# Autodesk Inventor assembly: Servo-Arm-52mm-Ball-Joint
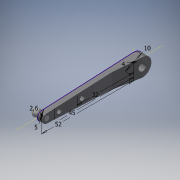
[picture p0: Inventor's stored thumbnail of the model, 180x180]
Saved by Autodesk Inventor 2018.2 (Build 222227000, 227)
## iProperties
Created: 2018-02-18
Part Number: Servo-Arm-52mm-Ball-Joint
Material: Generisch
Document SubType Name: Assembly
Designer: JochenAlt
Author: JochenAlt
## Documents named in this file (3)
- D:\Projects\Donna\CAD\Servo-Arm-52mm-Ball-Joint.iam
- D:\Projects\Donna\CAD\Ball-Joint-male.ipt
- D:\Projects\Donna\CAD\Servo-Arm-52mm.ipt
## Components (2 placed, 2 different names)
1. ball joint:1 — Passend:1, Passend:2
2. ServoArm:2 — Passend:1, Passend:2, Passend:3, Passend:4, Passend:5, Passend:6
## Relationships (6: Mate 6)
- Passend:1 [Mate]: ball joint:1 ↔ ServoArm:2
- Passend:2 [Mate]: ball joint:1 ↔ ServoArm:2
- Passend:3 [Mate]: ServoArm:2
- Passend:4 [Mate]: ServoArm:2
- Passend:5 [Mate]: ServoArm:2
- Passend:6 [Mate]: ServoArm:2
